# Autodesk Inventor assembly: ICF34_70mmNipple
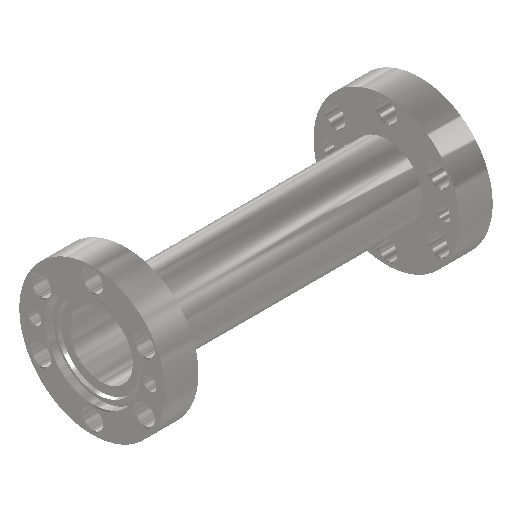
[picture p0: Inventor's stored thumbnail of the model, 512x512]
Saved by Autodesk Inventor 2026.2 (Build 302298000, 298)
## iProperties
Created: 2023-07-13
Part Number: ICF34_70mmNipple
Document SubType Name: Assembly
Designer: kuzmin
Author: kuzmin
## Documents named in this file (3)
- D:\repos\PIHTI\PALP\CF34-nipples-for-PALP\ICF34_70mmNipple.iam
- D:\repos\PIHTI\PALP\CF34-nipples-for-PALP\ICF34_70mmNipplePipe.ipt
- D:\repos\PIHTI\PALP\Prototype-PALP-CF34-flange.ipt
## Components (3 placed, 2 different names)
1. ICF34_70mmNipplePipe:1 — リジッド:1, 回転:3
2. Prototype-PALP-CF34-flange:1 — リジッド:1, メイト:1
3. Prototype-PALP-CF34-flange:2 — 回転:3, メイト:1
## Relationships (3: WeldJoint 1, RevoluteJoint 1, Mate 1)
- リジッド:1 [WeldJoint]: ICF34_70mmNipplePipe:1 ↔ Prototype-PALP-CF34-flange:1
- 回転:3 [RevoluteJoint]: ICF34_70mmNipplePipe:1 ↔ Prototype-PALP-CF34-flange:2
- メイト:1 [Mate]: Prototype-PALP-CF34-flange:1 ↔ Prototype-PALP-CF34-flange:2
